# Autodesk Inventor assembly: AutoArm
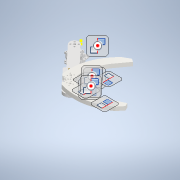
[picture p0: Inventor's stored thumbnail of the model, 180x180]
Saved by Autodesk Inventor 2020 (Build 240168000, 168)
## iProperties
Created: 2020-01-22
Part Number: AutoArm
Document SubType Name: Assembly
Designer: tdmp4
Author: tdmp4
## Documents named in this file (7)
- C:\Users\tdmp4\OneDrive\Documents\GitHub\CAD-2020\AutoArm.iam
- C:\Users\tdmp4\OneDrive\Documents\GitHub\CAD-2020\ServoCity\Servo Block.iam
- C:\Users\tdmp4\OneDrive\Documents\GitHub\CAD-2020\Autoarm parts\Claw arm.ipt
- C:\Users\tdmp4\OneDrive\Documents\GitHub\CAD-2020\RevRobotics\REV-41-1097.ipt
- C:\Users\tdmp4\OneDrive\Documents\GitHub\CAD-2020\Autoarm parts\REV-41-1363.ipt
- C:\Users\tdmp4\OneDrive\Documents\GitHub\CAD-2020\Autoarm parts\Spur Gear15.ipt
- C:\Users\tdmp4\OneDrive\Documents\GitHub\CAD-2020\Autoarm parts\Spur Gear15_MIR.ipt
## Components (6 placed, 6 different names)
1. Servo Block:1 [sub-assembly] — Mate:1, Mate:7
2. Claw arm:1 — Mate:1, Flush:1, Mate:4, Tangent:1, Mate:7, Mate:10
3. REV-41-1097:1 — Flush:1, Mate:4, Tangent:1, Mate:5, Mate:6
4. REV-41-1363:1 — Mate:5, Mate:6, Mate:8, Mate:9
5. Spur Gear1:1 — Mate:8, Mate:9, Flush:2
6. Spur Gear15_MIR:1 — Flush:2, Mate:10
## Relationships (11: Mate 8, Flush 2, Tangent 1)
- Mate:1: Servo Block:1 ↔ Claw arm:1
- Flush:1: Claw arm:1 ↔ REV-41-1097:1
- Mate:4: Claw arm:1 ↔ REV-41-1097:1
- Tangent:1: Claw arm:1 ↔ REV-41-1097:1
- Mate:5: REV-41-1097:1 ↔ REV-41-1363:1
- Mate:6: REV-41-1097:1 ↔ REV-41-1363:1
- Mate:7: Servo Block:1 ↔ Claw arm:1
- Mate:8: REV-41-1363:1 ↔ Spur Gear1:1
- Mate:9: REV-41-1363:1 ↔ Spur Gear1:1
- Flush:2: Spur Gear1:1 ↔ Spur Gear15_MIR:1
- Mate:10: Claw arm:1 ↔ Spur Gear15_MIR:1
